# Autodesk Inventor assembly: E000-Compresseur
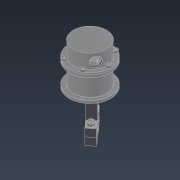
[picture p0: Inventor's stored thumbnail of the model, 180x180]
Saved by Autodesk Inventor 2021.3 (Build 253353000, 353)
## iProperties
Created: 2022-03-31
Part Number: E000-Compresseur
Document SubType Name: Assembly
Designer: remi
Author: remi
## Documents named in this file (5)
- C:\Users\remi\OneDrive\Documents\Cours\05-HEVS\S2fb\mechanic\CCo\project\Compressor\E000-Compresseur.iam
- C:\Users\remi\OneDrive\Documents\Cours\05-HEVS\S2fb\mechanic\CCo\project\Compressor\E001-Chambre.iam
- C:\Users\remi\OneDrive\Documents\Cours\05-HEVS\S2fb\mechanic\CCo\project\Compressor\E002-Piston.iam
- C:\Users\remi\OneDrive\Documents\Cours\05-HEVS\S2fb\mechanic\CCo\project\Compressor\E005-Bielle.iam
- C:\Users\remi\OneDrive\Documents\Inventor\Content Center Files\R2021\en-US\Bearing GB_T 5800-2003\Rolling bearing GB_T 5800-2003 -639_3.ipt
## Components (4 placed, 4 different names)
1. E001-Chambre:1 [sub-assembly] — Mate:1
2. E002-Piston:1 [sub-assembly] — Mate:1, Mate:2, Mate:3
3. E005-Bielle:1 [sub-assembly] — Mate:2
4. Bearing GB/T 5800-2003 639/3:1 — Mate:3
## Relationships (3: Mate 3)
- Mate:1: E001-Chambre:1 ↔ E002-Piston:1
- Mate:2: E002-Piston:1 ↔ E005-Bielle:1
- Mate:3: E002-Piston:1 ↔ Bearing GB/T 5800-2003 639/3:1
